# Autodesk Inventor assembly: UntererRührer
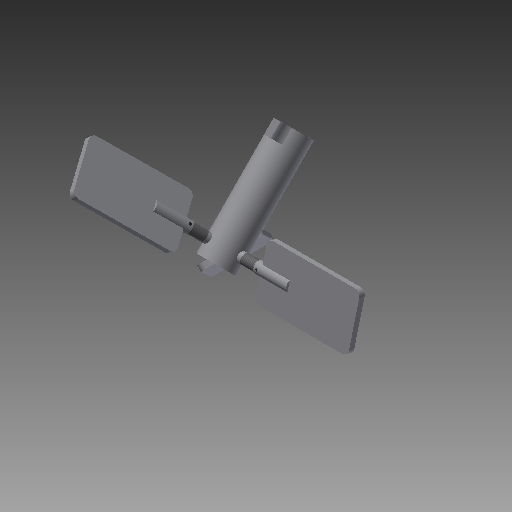
[picture p0: Inventor's stored thumbnail of the model, 512x512]
Saved by Autodesk Inventor 2017 (Build 210142000, 142)
## iProperties
Created: 2019-06-21
Part Number: UntererRührer
Document SubType Name: Assembly
Designer: Ole Simmering
Author: Ole Simmering
## Documents named in this file (4)
- C:\Users\Ole Simmering\Documents\GitHub\3D_modeling\Konstruktion und Apparatebau\HA5-Rührreaktor\Transfer\UntererRührer.iam
- C:\Users\Ole Simmering\Documents\GitHub\3D_modeling\Konstruktion und Apparatebau\HA5-Rührreaktor\Transfer\UntererRührerHalter.ipt
- C:\Users\Ole Simmering\Documents\GitHub\3D_modeling\Konstruktion und Apparatebau\HA5-Rührreaktor\Transfer\UntererRührerBlatt.ipt
- C:\Users\Ole Simmering\Documents\GitHub\3D_modeling\Konstruktion und Apparatebau\HA5-Rührreaktor\Transfer\Radial Pin Connection1.iam
## Components (7 placed, 3 different names)
1. UntererRührerHalter:1 — Mate:1, Mate:2
2. UntererRührerBlatt:1 — Mate:1, Mate:2
3. UntererRührerBlatt:2
4. UntererRührerBlatt:3 — Mate:3, Mate:4
5. Radial Pin Connection:1 [sub-assembly] — Mate:3, Mate:4
6. Radial Pin Connection:2 [sub-assembly]
7. Radial Pin Connection:3 [sub-assembly]
## Component patterns: (3 elements, first: UntererRührerBlatt:1), (3 elements, first: Radial Pin Connection:1)
## Relationships (4: Mate 4)
- Mate:1: UntererRührerHalter:1 ↔ UntererRührerBlatt:1
- Mate:2: UntererRührerHalter:1 ↔ UntererRührerBlatt:1
- Mate:3: UntererRührerBlatt:3 ↔ Radial Pin Connection:1
- Mate:4: UntererRührerBlatt:3 ↔ Radial Pin Connection:1
